# Autodesk Inventor assembly: Project Frame final
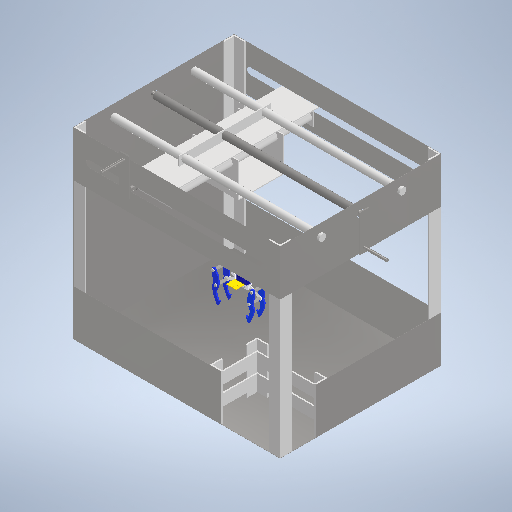
[picture p0: Inventor's stored thumbnail of the model, 512x512]
Saved by Autodesk Inventor 2025.2 (Build 292293000, 293)
## iProperties
Created: 2025-02-04
Part Number: Project Frame final
Document SubType Name: Assembly
Designer: Khushal
Author: Khushal
## Documents named in this file (16)
- C:\Users\Khushal\Documents\College\Sem 4\TA212\Project_Latest\Project Assembly final.iam
- C:\Users\Khushal\Documents\College\Sem 4\TA212\Project_Latest\project base plate.ipt
- C:\Users\Khushal\Documents\College\Sem 4\TA212\Project_Latest\project MS angle.ipt
- C:\Users\Khushal\Documents\College\Sem 4\TA212\Project_Latest\project Backrestfinal.ipt
- C:\Users\Khushal\Documents\College\Sem 4\TA212\Project_Latest\project slot.iam
- C:\Users\Khushal\Documents\College\Sem 4\TA212\Project_Latest\project support plate small.ipt
- C:\Users\Khushal\Documents\College\Sem 4\TA212\Project_Latest\project side supporting plate.ipt
- C:\Users\Khushal\Documents\College\Sem 4\TA212\Project_Latest\project slit.ipt
- C:\Users\Khushal\Documents\College\Sem 4\TA212\Project_Latest\project supporting plate.ipt
- C:\Users\Khushal\Documents\College\Sem 4\TA212\Project_Latest\project front supporting plate.ipt
- C:\Users\Khushal\Documents\College\Sem 4\TA212\Project\leadscrew_modified.ipt
- C:\Users\Khushal\Documents\College\Sem 4\TA212\Project\leadscrew_modified_long.ipt
- C:\Users\Khushal\Documents\College\Sem 4\TA212\Project\support rod.ipt
- C:\Users\Khushal\Documents\College\Sem 4\TA212\Project_Latest\Claw_Platform_2.ipt
- C:\Users\Khushal\Documents\College\Sem 4\TA212\Project\motor holder.ipt
- C:\Users\Khushal\Documents\College\Sem 4\TA212\Gripper_1\robotic-gripper-18.snapshot.4\Autodesk Inventor\_Robotic Gripper Assembly.iam
## Components (20 placed, 15 different names)
1. project base plate:1 — Mate:1, Rigid:1, Mate:2, Mate:3, Mate:4, Rigid:2, Rigid:3, Rigid:4, Mate:11
2. project MS angle:1 — Mate:3, Rigid:3, Mate:8, Mate:13, Rigid:10, Mate:15, Rigid:12, Rigid:14, Rigid:15
3. project MS angle:2 — Mate:1, Rigid:1, Mate:12, Rigid:9
4. project MS angle:3 — Mate:4, Rigid:2, Rigid:6, Mate:16, Rigid:13
5. project MS angle:4 — Mate:2, Rigid:4, Mate:6, Mate:17
6. project Backrestfinal:1 — Mate:6, Rigid:6, Insert:2, Insert:4, Insert:5
7. project side supporting plate:1 — Mate:8, Mate:9, Rigid:14
8. project slot:1 [sub-assembly] — Mate:9, Mate:11
9. project slit:1 — Mate:12, Rigid:9
10. project support plate small:1 — Mate:13, Rigid:10
11. project supporting plate:2 — Mate:15, Rigid:12
12. project front supporting plate:1 — Mate:16, Rigid:13
13. leadscrew_modified_long:1 — Insert:2
14. project slit:2 — Mate:17, Rigid:15
15. support rod:1 — Insert:4, Insert:6
16. support rod:2 — Insert:5
17. Claw_Platform_2:1 — Insert:6, Insert:7
18. leadscrew_modified:1 — Insert:7, Insert:8
19. motor holder:1 — Insert:8, Mate:18
20. _Robotic Gripper Assembly:1 [sub-assembly] — Mate:18
## Relationships (31: Mate 14, WeldJoint 11, Insert 6)
- Mate:1: project base plate:1 ↔ project MS angle:2
- Rigid:1 [WeldJoint]: project base plate:1 ↔ project MS angle:2
- Mate:2: project base plate:1 ↔ project MS angle:4
- Mate:3: project base plate:1 ↔ project MS angle:1
- Mate:4: project base plate:1 ↔ project MS angle:3
- Rigid:2 [WeldJoint]: project base plate:1 ↔ project MS angle:3
- Rigid:3 [WeldJoint]: project base plate:1 ↔ project MS angle:1
- Rigid:4 [WeldJoint]: project base plate:1 ↔ project MS angle:4
- Mate:6: project MS angle:4 ↔ project Backrestfinal:1
- Rigid:6 [WeldJoint]: project MS angle:3 ↔ project Backrestfinal:1
- Mate:8: project MS angle:1 ↔ project side supporting plate:1
- Mate:9: project side supporting plate:1 ↔ project slot:1
- Mate:11: project base plate:1 ↔ project slot:1
- Mate:12: project MS angle:2 ↔ project slit:1
- Rigid:9 [WeldJoint]: project MS angle:2 ↔ project slit:1
- Mate:13: project MS angle:1 ↔ project support plate small:1
- Rigid:10 [WeldJoint]: project MS angle:1 ↔ project support plate small:1
- Mate:15: project MS angle:1 ↔ project supporting plate:2
- Rigid:12 [WeldJoint]: project MS angle:1 ↔ project supporting plate:2
- Mate:16: project MS angle:3 ↔ project front supporting plate:1
- Rigid:13 [WeldJoint]: project MS angle:3 ↔ project front supporting plate:1
- Rigid:14 [WeldJoint]: project MS angle:1 ↔ project side supporting plate:1
- Insert:2 (5 mm): project Backrestfinal:1 ↔ leadscrew_modified_long:1
- Mate:17: project MS angle:4 ↔ project slit:2
- Rigid:15 [WeldJoint]: project MS angle:1 ↔ project slit:2
- Insert:4 (-5 mm): project Backrestfinal:1 ↔ support rod:1
- Insert:5 (-5 mm): project Backrestfinal:1 ↔ support rod:2
- Insert:6 (-300 mm): support rod:1 ↔ Claw_Platform_2:1
- Insert:7 (-15 mm): Claw_Platform_2:1 ↔ leadscrew_modified:1
- Insert:8 (-250 mm): leadscrew_modified:1 ↔ motor holder:1
- Mate:18 (175 mm): motor holder:1 ↔ _Robotic Gripper Assembly:1
